# Autodesk Inventor assembly: OBG-Dribbler und Chipper
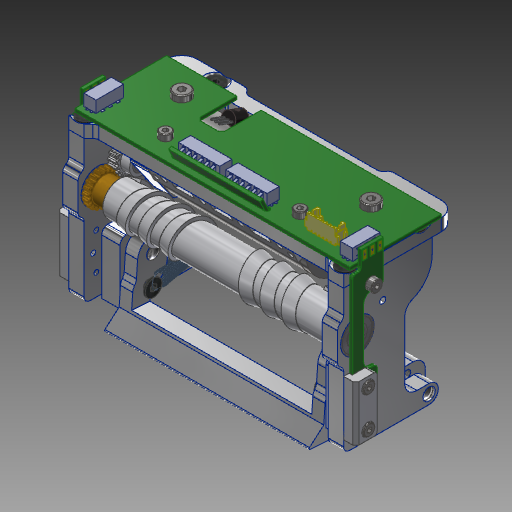
[picture p0: Inventor's stored thumbnail of the model, 512x512]
Saved by Autodesk Inventor 2019.4 (Build 234330000, 330)
## iProperties
Part Number: OBG-Dribbler und Chipper
Material: Generisch
Document SubType Name: Assembly
Designer: rYan
Mass: 268.659 g
Surface Area: 545.327 cm^2
Volume: 68.049 cm^3
Density: 3.94802 g/cm^3
Author: rYan
## Documents named in this file (3)
- D:\TIGERsGIT\Hardware\mechanik\2020\Inventor\Robot\Dribbler\OBG-Dribbler und Chipper.iam
- D:\TIGERsGIT\Hardware\mechanik\2020\Inventor\Robot\Dribbler\UBG-Dribbler.iam
- D:\TIGERsGIT\Hardware\mechanik\2020\Inventor\Robot\Dribbler\UBG-Dribblerhalter.iam
## Components (2 placed, 2 different names)
1. UBG-Dribbler:1 [sub-assembly] — Passend:1, Passend:5, Winkel:1
2. UBG-Dribblerhalter:1 [sub-assembly] — Passend:3, Fluchtend:1, Passend:4, Passend:5, Winkel:1
## Relationships (6: Mate 4, Flush 1, Angle 1)
- Passend:1 [Mate]: UBG-Dribbler:1
- Passend:3 [Mate]: UBG-Dribblerhalter:1
- Fluchtend:1 [Flush]: UBG-Dribblerhalter:1
- Passend:4 [Mate]: UBG-Dribblerhalter:1
- Passend:5 [Mate]: UBG-Dribbler:1 ↔ UBG-Dribblerhalter:1
- Winkel:1 [Angle] (0 deg): UBG-Dribbler:1 ↔ UBG-Dribblerhalter:1
